# Autodesk Inventor assembly: Arm 2.0 Assembly
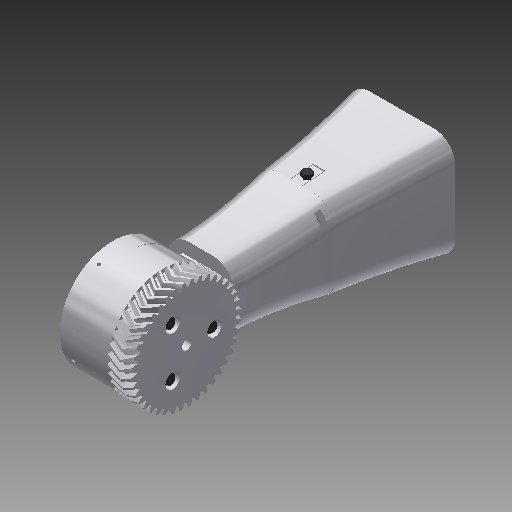
[picture p0: Inventor's stored thumbnail of the model, 512x512]
Saved by Autodesk Inventor 2017 (Build 210142000, 142)
## iProperties
Created: 2017-09-28
Part Number: Arm 2.0 Assembly
Document SubType Name: Assembly
Designer: Zach
Author: Zach
## Documents named in this file (18)
- C:\Users\Dell\Documents\GitHub\tr1\src\Body\Arm Assembly\Forearm Assembly\Forearm Assembly.iam
- C:\Users\Dell\Documents\GitHub\tr1\lib\12V DC Motor 378-1.ipt
- C:\Users\Dell\Documents\GitHub\tr1\lib\8mm Hub.ipt
- C:\Users\Dell\Documents\GitHub\tr1\src\Body\Arm Assembly\Forearm Assembly\AA036.ipt
- C:\Users\Dell\Documents\GitHub\tr1\src\Body\Arm Assembly\Forearm Assembly\AA037.ipt
- C:\Users\Dell\Documents\GitHub\tr1\src\Body\Arm Assembly\Forearm Assembly\AA016b.ipt
- C:\Users\Dell\Documents\GitHub\tr1\src\Body\Arm Assembly\Arm Assembly\Design Accelerator\Spur Gears12.iam
- C:\Users\Dell\Documents\GitHub\tr1\src\Body\Arm Assembly\Forearm Assembly\AA041.ipt
- C:\Users\Dell\Documents\GitHub\tr1\lib\Content Center Files\R2017\en-US\ISO 7045  H\ISO 7045 - M3 x 8 - 4.8 - H - ISO.ipt
- C:\Users\Dell\Documents\GitHub\tr1\lib\Content Center Files\R2017\en-US\ISO 4018\ISO 4018 - M5 x 25.ipt
- C:\Users\Dell\Documents\GitHub\tr1\lib\Content Center Files\R2017\en-US\ISO 4035(2)\ISO 4035 - M5 - ISO.ipt
- C:\Users\Dell\Documents\GitHub\tr1\lib\Content Center Files\R2017\en-US\ISO 4018\ISO 4018 - M5 x 35.ipt
- C:\Users\Dell\Documents\GitHub\tr1\lib\EMS22XXX-D28-LSX.ipt
- C:\Users\Dell\Documents\GitHub\tr1\src\Body\Arm Assembly\Forearm Assembly\AA051.ipt
- C:\Users\Dell\Documents\GitHub\tr1\lib\6mm x 120mm D Shaft.ipt
- C:\Users\Dell\Documents\GitHub\tr1\lib\6mm Mounting Hub, thin.ipt
- C:\Users\Dell\Documents\GitHub\tr1\src\Body\Arm Assembly\Forearm Assembly\AASG03b.ipt
- C:\Users\Dell\Documents\GitHub\tr1\lib\Content Center Files\R2017\en-US\ISO 7045  H\ISO 7045 - M3 x 12 - 4.8 - H - ISO.ipt
## Components (39 placed, 17 different names)
1. AA016b:1 — Mate:518, Mate:519, Mate:520, Mate:530, Mate:664, Mate:665, Mate:671, Mate:673, Mate:675, Mate:676, Mate:677, Mate:877, Mate:878, Mate:1206, Mate:1207, Angle:26
2. AA036:1 — Mate:501, Mate:502, Mate:698, Mate:868, Mate:871, Mate:872, Mate:939, Mate:1197, Mate:1198, Mate:1199, Mate:1200, Mate:1330, Mate:1332
3. AA037:1 — Mate:501, Mate:502, Mate:514, Mate:515, Mate:516, Mate:518, Mate:519, Mate:520, Mate:530, Mate:664, Mate:665, Mate:698, Mate:866, Mate:867, Mate:873, Mate:874, Mate:875, Mate:876, Flush:25, Flush:26, Mate:1338, Mate:1339, Mate:1340, Mate:1341, Mate:1360, Mate:1361, Mate:1362, Mate:1363
4. AA041:1 — Mate:675, Mate:676, Mate:677, Mate:682, Mate:683, Mate:684, Mate:685
5. AA051:1 — Mate:1197, Mate:1335
6. 12V DC Motor 378-1:4 — Mate:514, Mate:515, Mate:516, Mate:1292, Mate:1303, Mate:1304
7. 8mm Hub:14 — Mate:1198, Mate:1199, Mate:1200, Mate:1335, Mate:1342, Mate:1343, Mate:1344, Mate:1345, Mate:1346, Mate:1347
8. 6mm x 120mm D Shaft:1 — Mate:1292, Mate:1303, Mate:1304, Mate:1305, Mate:1318, Mate:1336
9. EMS22XXX-D28-LSX:5 — Mate:1206, Mate:1207, Angle:26, Mate:1210, Mate:1316, Mate:1326
10. AASG08 [sub-assembly] — Mate:671, Mate:673, Mate:680, Mate:681, Mate:1305, Mate:1317, Mate:1319, Mate:1326, Mate:1348, Mate:1350, Mate:1351, Mate:1352, Mate:1353, Mate:1354, Mate:1355, Mate:1356, Mate:1357, Mate:1358, Mate:1359
11. ISO 7045 H M3 x 8 - 4.8 - H:1 — Mate:680, Mate:681
12. ISO 7045 H M3 x 8 - 4.8 - H:2 — Mate:682, Mate:685
13. ISO 7045 H M3 x 8 - 4.8 - H:3 — Mate:683, Mate:684
14. ISO 4035 M5:3 — Mate:869, Mate:872
15. ISO 4035 M5:4 — Mate:870, Mate:871
16. ISO 4018 M5 x 25:33 — Mate:939, Mate:1329, Mate:1334
17. ISO 4018 M5 x 25:34 — Mate:1327, Mate:1331
18. ISO 4018 M5 x 25:35 — Mate:1328, Mate:1333
19. ISO 4018 M5 x 25:36 — Mate:876, Mate:878
20. ISO 4018 M5 x 25:37 — Mate:875, Mate:877
21. ISO 4018 M5 x 25:38 — Mate:874, Flush:26
22. ISO 4018 M5 x 25:39 — Mate:873, Flush:25
23. ISO 4018 M5 x 35:1 — Mate:866, Mate:867, Flush:24, Mate:869
24. ISO 4018 M5 x 35:2 — Mate:868, Flush:24, Mate:870
25. 6mm Mounting Hub, thin:2 — Mate:1316, Mate:1317, Mate:1210, Mate:1354
26. 6mm Mounting Hub, thin:3 — Mate:1318, Mate:1319, Mate:1349
27. Spur Gear2:1 — Mate:1327, Mate:1328, Mate:1329, Mate:1330, Mate:1331, Mate:1332, Mate:1333, Mate:1334, Mate:1337
28. ISO 4018 M5 x 35:3 — Mate:1338, Mate:1339
29. ISO 4018 M5 x 35:4 — Mate:1340, Mate:1341
30. ISO 7045 H M3 x 12 - 4.8 - H:1 — Mate:1345, Mate:1347
31. ISO 7045 H M3 x 12 - 4.8 - H:2 — Mate:1342, Mate:1343
32. ISO 7045 H M3 x 12 - 4.8 - H:3 — Mate:1344, Mate:1346
33. ISO 7045 H M3 x 8 - 4.8 - H:4 — Mate:1348, Mate:1349, Mate:1350
34. ISO 7045 H M3 x 8 - 4.8 - H:5 — Mate:1351, Mate:1352
35. ISO 7045 H M3 x 8 - 4.8 - H:6 — Mate:1353, Mate:1355
36. ISO 7045 H M3 x 8 - 4.8 - H:7 — Mate:1358, Mate:1359
37. ISO 7045 H M3 x 8 - 4.8 - H:8 — Mate:1356, Mate:1357
38. ISO 7045 H M3 x 8 - 4.8 - H:9 — Mate:1360, Mate:1362
39. ISO 7045 H M3 x 8 - 4.8 - H:10 — Mate:1361, Mate:1363
## Relationships (94: Mate 90, Flush 3, Angle 1)
- Mate:501: AA036:1 ↔ AA037:1
- Mate:502: AA036:1 ↔ AA037:1
- Mate:514: AA037:1 ↔ 12V DC Motor 378-1:4
- Mate:515: AA037:1 ↔ 12V DC Motor 378-1:4
- Mate:516: AA037:1 ↔ 12V DC Motor 378-1:4
- Mate:518: AA016b:1 ↔ AA037:1
- Mate:519: AA016b:1 ↔ AA037:1
- Mate:520: AA016b:1 ↔ AA037:1
- Mate:530: AA016b:1 ↔ AA037:1
- Mate:664: AA016b:1 ↔ AA037:1
- Mate:665: AA016b:1 ↔ AA037:1
- Mate:671: AA016b:1 ↔ AASG08
- Mate:673: AA016b:1 ↔ AASG08
- Mate:675: AA016b:1 ↔ AA041:1
- Mate:676: AA016b:1 ↔ AA041:1
- Mate:677: AA016b:1 ↔ AA041:1
- Mate:680: AASG08 ↔ ISO 7045 H M3 x 8 - 4.8 - H:1
- Mate:681: AASG08 ↔ ISO 7045 H M3 x 8 - 4.8 - H:1
- Mate:682: AA041:1 ↔ ISO 7045 H M3 x 8 - 4.8 - H:2
- Mate:683: AA041:1 ↔ ISO 7045 H M3 x 8 - 4.8 - H:3
- Mate:684: AA041:1 ↔ ISO 7045 H M3 x 8 - 4.8 - H:3
- Mate:685: AA041:1 ↔ ISO 7045 H M3 x 8 - 4.8 - H:2
- Mate:698: AA036:1 ↔ AA037:1
- Mate:866: AA037:1 ↔ ISO 4018 M5 x 35:1
- Mate:867: AA037:1 ↔ ISO 4018 M5 x 35:1
- Mate:868: AA036:1 ↔ ISO 4018 M5 x 35:2
- Flush:24: ISO 4018 M5 x 35:1 ↔ ISO 4018 M5 x 35:2
- Mate:869: ISO 4035 M5:3 ↔ ISO 4018 M5 x 35:1
- Mate:870: ISO 4035 M5:4 ↔ ISO 4018 M5 x 35:2
- Mate:871: AA036:1 ↔ ISO 4035 M5:4
- Mate:872: AA036:1 ↔ ISO 4035 M5:3
- Mate:873: AA037:1 ↔ ISO 4018 M5 x 25:39
- Mate:874: AA037:1 ↔ ISO 4018 M5 x 25:38
- Mate:875: AA037:1 ↔ ISO 4018 M5 x 25:37
- Mate:876: AA037:1 ↔ ISO 4018 M5 x 25:36
- Flush:25 (-9 mm): AA037:1 ↔ ISO 4018 M5 x 25:39
- Flush:26 (9 mm): AA037:1 ↔ ISO 4018 M5 x 25:38
- Mate:877: AA016b:1 ↔ ISO 4018 M5 x 25:37
- Mate:878: AA016b:1 ↔ ISO 4018 M5 x 25:36
- Mate:939: AA036:1 ↔ ISO 4018 M5 x 25:33
- Mate:1197: AA036:1 ↔ AA051:1
- Mate:1198: AA036:1 ↔ 8mm Hub:14
- Mate:1199: AA036:1 ↔ 8mm Hub:14
- Mate:1200: AA036:1 ↔ 8mm Hub:14
- Mate:1206: AA016b:1 ↔ EMS22XXX-D28-LSX:5
- Mate:1207: AA016b:1 ↔ EMS22XXX-D28-LSX:5
- Angle:26 (180 deg): AA016b:1 ↔ EMS22XXX-D28-LSX:5
- Mate:1210: EMS22XXX-D28-LSX:5 ↔ 6mm Mounting Hub, thin:2
- Mate:1292: 12V DC Motor 378-1:4 ↔ 6mm x 120mm D Shaft:1
- Mate:1303: 12V DC Motor 378-1:4 ↔ 6mm x 120mm D Shaft:1
- Mate:1304: 12V DC Motor 378-1:4 ↔ 6mm x 120mm D Shaft:1
- Mate:1305: 6mm x 120mm D Shaft:1 ↔ AASG08
- Mate:1316: EMS22XXX-D28-LSX:5 ↔ 6mm Mounting Hub, thin:2
- Mate:1317: AASG08 ↔ 6mm Mounting Hub, thin:2
- Mate:1318: 6mm x 120mm D Shaft:1 ↔ 6mm Mounting Hub, thin:3
- Mate:1319: AASG08 ↔ 6mm Mounting Hub, thin:3
- Mate:1326: EMS22XXX-D28-LSX:5 ↔ AASG08
- Mate:1327: ISO 4018 M5 x 25:34 ↔ Spur Gear2:1
- Mate:1328: ISO 4018 M5 x 25:35 ↔ Spur Gear2:1
- Mate:1329: ISO 4018 M5 x 25:33 ↔ Spur Gear2:1
- Mate:1330: AA036:1 ↔ Spur Gear2:1
- Mate:1331: ISO 4018 M5 x 25:34 ↔ Spur Gear2:1
- Mate:1332: AA036:1 ↔ Spur Gear2:1
- Mate:1333: ISO 4018 M5 x 25:35 ↔ Spur Gear2:1
- Mate:1334: ISO 4018 M5 x 25:33 ↔ Spur Gear2:1
- Mate:1335: AA051:1 ↔ 8mm Hub:14
- Mate:1336: 6mm x 120mm D Shaft:1
- Mate:1337: Spur Gear2:1
- Mate:1338: AA037:1 ↔ ISO 4018 M5 x 35:3
- Mate:1339: AA037:1 ↔ ISO 4018 M5 x 35:3
- Mate:1340: AA037:1 ↔ ISO 4018 M5 x 35:4
- Mate:1341: AA037:1 ↔ ISO 4018 M5 x 35:4
- Mate:1342: 8mm Hub:14 ↔ ISO 7045 H M3 x 12 - 4.8 - H:2
- Mate:1343: 8mm Hub:14 ↔ ISO 7045 H M3 x 12 - 4.8 - H:2
- Mate:1344: 8mm Hub:14 ↔ ISO 7045 H M3 x 12 - 4.8 - H:3
- Mate:1345: 8mm Hub:14 ↔ ISO 7045 H M3 x 12 - 4.8 - H:1
- Mate:1346: 8mm Hub:14 ↔ ISO 7045 H M3 x 12 - 4.8 - H:3
- Mate:1347: 8mm Hub:14 ↔ ISO 7045 H M3 x 12 - 4.8 - H:1
- Mate:1348: AASG08 ↔ ISO 7045 H M3 x 8 - 4.8 - H:4
- Mate:1349: 6mm Mounting Hub, thin:3 ↔ ISO 7045 H M3 x 8 - 4.8 - H:4
- Mate:1350: AASG08 ↔ ISO 7045 H M3 x 8 - 4.8 - H:4
- Mate:1351: AASG08 ↔ ISO 7045 H M3 x 8 - 4.8 - H:5
- Mate:1352: AASG08 ↔ ISO 7045 H M3 x 8 - 4.8 - H:5
- Mate:1353: AASG08 ↔ ISO 7045 H M3 x 8 - 4.8 - H:6
- Mate:1354: AASG08 ↔ 6mm Mounting Hub, thin:2
- Mate:1355: AASG08 ↔ ISO 7045 H M3 x 8 - 4.8 - H:6
- Mate:1356: AASG08 ↔ ISO 7045 H M3 x 8 - 4.8 - H:8
- Mate:1357: AASG08 ↔ ISO 7045 H M3 x 8 - 4.8 - H:8
- Mate:1358: AASG08 ↔ ISO 7045 H M3 x 8 - 4.8 - H:7
- Mate:1359: AASG08 ↔ ISO 7045 H M3 x 8 - 4.8 - H:7
- Mate:1360: AA037:1 ↔ ISO 7045 H M3 x 8 - 4.8 - H:9
- Mate:1361: AA037:1 ↔ ISO 7045 H M3 x 8 - 4.8 - H:10
- Mate:1362: AA037:1 ↔ ISO 7045 H M3 x 8 - 4.8 - H:9
- Mate:1363: AA037:1 ↔ ISO 7045 H M3 x 8 - 4.8 - H:10
